# Autodesk Inventor assembly: Practice Assemble
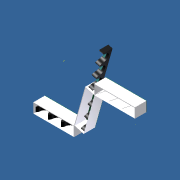
[picture p0: Inventor's stored thumbnail of the model, 180x180]
Saved by Autodesk Inventor 2012 (Build 160160000, 160)
## iProperties
Created: 2012-02-03
Part Number: Practice Assemble
Document SubType Name: Assembly
Designer: Allison Garza
Author: Allison Garza
## Documents named in this file (13)
- C:\Users\Allison Garza\Documents\Rice Spring 2012\MRSL\Practice Assemble.iam
- C:\Users\Allison Garza\Documents\Rice Spring 2012\MRSL\circuit board 2.ipt
- C:\Users\Allison Garza\Documents\Rice Spring 2012\MRSL\side panel.ipt
- C:\Users\Allison Garza\Documents\Rice Spring 2012\MRSL\bottom panel.ipt
- C:\Users\Allison Garza\Documents\Rice Spring 2012\MRSL\end panel.ipt
- C:\Users\Allison Garza\Documents\Rice Spring 2012\MRSL\top panel for hinge.ipt
- C:\Users\Allison Garza\Documents\Rice Spring 2012\MRSL\side panel for hinge.ipt
- C:\Users\Allison Garza\Documents\Rice Spring 2012\MRSL\top panel for hinge left.ipt
- C:\Users\Allison Garza\Documents\Rice Spring 2012\MRSL\Hinge Assembly.iam
- C:\Users\Allison Garza\Documents\Rice Spring 2012\MRSL\bottom panel right.ipt
- C:\Users\Allison Garza\Documents\Rice Spring 2012\MRSL\top panel normal.ipt
- C:\Users\Allison Garza\Documents\Rice Spring 2012\MRSL\bottom panel left.ipt
- C:\Users\Allison Garza\Documents\Rice Spring 2012\MRSL\Swirly Assembly.iam
## Components (20 placed, 12 different names)
1. circuit board 2:1 — Mate:5, Flush:3, Flush:4, Mate:10, Flush:8, Mate:11, Mate:36, Mate:46, Flush:24, Mate:62, Mate:64
2. side panel:2 — Mate:5, Flush:3, Flush:4
3. end panel:1 — Mate:10, Flush:8, Flush:9, Mate:12, Mate:37, Flush:16, Mate:63
4. top panel for hinge:1 — Flush:9, Mate:11, Mate:12, Mate:23, Mate:24, Mate:26, Mate:46, Flush:24
5. Swirly Assembly:1 [sub-assembly] — Mate:62, Mate:63, Mate:64
6. circuit board 2:1 — Mate:18, Flush:11, Mate:20, Flush:12, Flush:13, Mate:21, Flush:14, Mate:34, Flush:15, Mate:65, Mate:67
7. Swirly Assembly:2 [sub-assembly] — Mate:65, Mate:66, Mate:67
8. side panel for hinge:1 — Mate:18, Flush:11, Mate:35, Mate:66, Flush:26
9. side panel for hinge:2 — Mate:20, Flush:12, Flush:13, Mate:22, Mate:69
10. top panel for hinge left:1 — Mate:21, Mate:22, Flush:14, Mate:28, Mate:29, Mate:31, Mate:33, Flush:26
11. Hinge Assembly:1 [sub-assembly] — Mate:23, Mate:24, Mate:25, Mate:28, Mate:30, Mate:32
12. bottom panel:2 — Mate:34, Mate:35, Flush:15, Mate:51, Mate:52, Mate:56, Mate:57, Mate:58
13. bottom panel right:1 — Mate:36, Mate:37, Flush:16
14. circuit board 2:3 — Mate:40, Flush:18, Flush:19, Mate:41, Flush:20, Flush:21, Mate:42, Flush:22, Mate:48, Mate:68, Mate:70
15. Swirly Assembly:3 [sub-assembly] — Mate:68, Mate:69, Mate:70
16. side panel for hinge:3 — Mate:40, Flush:18, Flush:19, Mate:43, Mate:47, Flush:25
17. end panel:2 — Mate:41, Flush:20, Flush:21
18. top panel normal:1 — Mate:42, Mate:43, Flush:22
19. bottom panel left:1 — Mate:47, Flush:25, Mate:48, Mate:59, Mate:60, Mate:61
20. Hinge Assembly:2 [sub-assembly] — Mate:56, Mate:57, Mate:58, Mate:59, Mate:60, Mate:61
## Relationships (77: Mate 56, Flush 21)
- Mate:5: circuit board 2:1 ↔ side panel:2
- Flush:3: circuit board 2:1 ↔ side panel:2
- Flush:4: circuit board 2:1 ↔ side panel:2
- Mate:10: circuit board 2:1 ↔ end panel:1
- Flush:8: circuit board 2:1 ↔ end panel:1
- Flush:9: end panel:1 ↔ top panel for hinge:1
- Mate:11: circuit board 2:1 ↔ top panel for hinge:1
- Mate:12: end panel:1 ↔ top panel for hinge:1
- [Mate]: circuit board 2:1 ↔ Swirly Assembly:2
- [Flush] (3.175 mm): circuit board 2:1 ↔ Swirly Assembly:2
- [Mate]: circuit board 2:1 ↔ Swirly Assembly:2
- Mate:18: circuit board 2:1 ↔ side panel for hinge:1
- Flush:11: circuit board 2:1 ↔ side panel for hinge:1
- [Mate]: Swirly Assembly:2 ↔ side panel for hinge:1
- Mate:20: circuit board 2:1 ↔ side panel for hinge:2
- Flush:12: circuit board 2:1 ↔ side panel for hinge:2
- Flush:13: circuit board 2:1 ↔ side panel for hinge:2
- Mate:21: circuit board 2:1 ↔ top panel for hinge left:1
- Mate:22: side panel for hinge:2 ↔ top panel for hinge left:1
- Flush:14: circuit board 2:1 ↔ top panel for hinge left:1
- Mate:23: top panel for hinge:1 ↔ Hinge Assembly:1
- Mate:24: top panel for hinge:1 ↔ Hinge Assembly:1
- Mate:25: Hinge Assembly:1
- Mate:26: top panel for hinge:1
- Mate:27
- Mate:28: top panel for hinge left:1 ↔ Hinge Assembly:1
- Mate:29: top panel for hinge left:1
- Mate:30: Hinge Assembly:1
- Mate:31: top panel for hinge left:1
- Mate:32: Hinge Assembly:1
- Mate:33: top panel for hinge left:1
- Mate:34: circuit board 2:1 ↔ bottom panel:2
- Mate:35: side panel for hinge:1 ↔ bottom panel:2
- Flush:15: circuit board 2:1 ↔ bottom panel:2
- Mate:36: circuit board 2:1 ↔ bottom panel right:1
- Mate:37: end panel:1 ↔ bottom panel right:1
- Flush:16: end panel:1 ↔ bottom panel right:1
- [Mate]: circuit board 2:3 ↔ Swirly Assembly:3
- [Mate]: circuit board 2:3 ↔ Swirly Assembly:3
- [Flush] (3.175 mm): circuit board 2:3 ↔ Swirly Assembly:3
- Mate:40: circuit board 2:3 ↔ side panel for hinge:3
- Flush:18: circuit board 2:3 ↔ side panel for hinge:3
- Flush:19: circuit board 2:3 ↔ side panel for hinge:3
- Mate:41: circuit board 2:3 ↔ end panel:2
- Flush:20: circuit board 2:3 ↔ end panel:2
- Flush:21: circuit board 2:3 ↔ end panel:2
- Mate:42: circuit board 2:3 ↔ top panel normal:1
- Mate:43: side panel for hinge:3 ↔ top panel normal:1
- Flush:22: circuit board 2:3 ↔ top panel normal:1
- [Mate]: circuit board 2:1 ↔ Swirly Assembly:1
- [Mate]: circuit board 2:1 ↔ Swirly Assembly:1
- [Flush] (3.175 mm): circuit board 2:1 ↔ Swirly Assembly:1
- Mate:46: circuit board 2:1 ↔ top panel for hinge:1
- Flush:24: circuit board 2:1 ↔ top panel for hinge:1
- Mate:47: side panel for hinge:3 ↔ bottom panel left:1
- Flush:25: side panel for hinge:3 ↔ bottom panel left:1
- Mate:48: circuit board 2:3 ↔ bottom panel left:1
- Mate:51: bottom panel:2
- Mate:52: bottom panel:2
- Mate:54
- Mate:55
- Mate:56: bottom panel:2 ↔ Hinge Assembly:2
- Mate:57: bottom panel:2 ↔ Hinge Assembly:2
- Mate:58: bottom panel:2 ↔ Hinge Assembly:2
- Mate:59: bottom panel left:1 ↔ Hinge Assembly:2
- Mate:60: bottom panel left:1 ↔ Hinge Assembly:2
- Mate:61: bottom panel left:1 ↔ Hinge Assembly:2
- Mate:62: circuit board 2:1 ↔ Swirly Assembly:1
- Mate:63: end panel:1 ↔ Swirly Assembly:1
- Mate:64: circuit board 2:1 ↔ Swirly Assembly:1
- Mate:65: circuit board 2:1 ↔ Swirly Assembly:2
- Mate:66: Swirly Assembly:2 ↔ side panel for hinge:1
- Mate:67: circuit board 2:1 ↔ Swirly Assembly:2
- Mate:68: circuit board 2:3 ↔ Swirly Assembly:3
- Mate:69: side panel for hinge:2 ↔ Swirly Assembly:3
- Mate:70: circuit board 2:3 ↔ Swirly Assembly:3
- Flush:26: side panel for hinge:1 ↔ top panel for hinge left:1
